# Autodesk Inventor assembly: ABD_MX_64_Roll_Fixation_Set
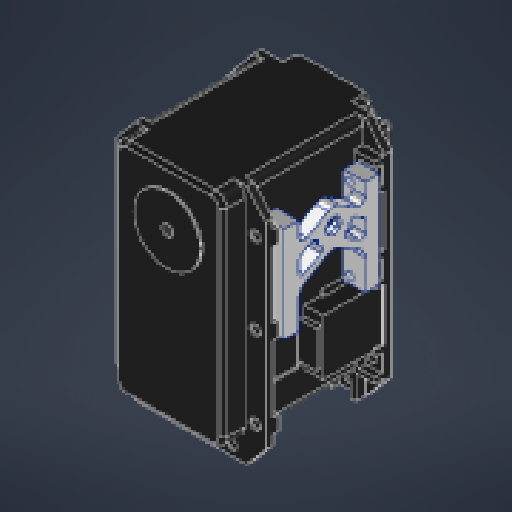
[picture p0: Inventor's stored thumbnail of the model, 512x512]
Saved by Autodesk Inventor 2024.3 (Build 283343000, 343)
## iProperties
Created: 2024-02-15
Part Number: ABD_MX_64_Roll_Fixation_Set
Document SubType Name: Assembly
Designer: ASUS
Author: ASUS
## Documents named in this file (4)
- C:\Users\ASUS\Desktop\Anti_Backlash_Structure_OP\v4_Frame\ABD_MX_64_Roll_Fixation_Set.iam
- C:\Users\ASUS\Desktop\Anti_Backlash_Structure_OP\v4_Frame\Roll_Fixation_L.ipt
- C:\Users\ASUS\Desktop\Anti_Backlash_Structure_OP\v4_Frame\Roll_Fixation_R.ipt
- C:\Users\ASUS\Desktop\Anti_Backlash_Structure_OP\ROBOTIS(Inventor 2024 ver.)\DXL\MX-106T.ipt
## Components (3 placed, 3 different names)
1. Roll_Fixation_R:1 — 플러쉬:1, 메이트:11, 메이트:19
2. Roll_Fixation_L:1 — 플러쉬:1, 메이트:12, 메이트:13, 메이트:14
3. MX-106T:1 — 메이트:11, 메이트:12, 메이트:13, 메이트:14, 메이트:19
## Relationships (6: Mate 5, Flush 1)
- 플러쉬:1 [Flush]: Roll_Fixation_R:1 ↔ Roll_Fixation_L:1
- 메이트:11 [Mate] (0.05 mm): Roll_Fixation_R:1 ↔ MX-106T:1
- 메이트:12 [Mate] (0.05 mm): Roll_Fixation_L:1 ↔ MX-106T:1
- 메이트:13 [Mate]: Roll_Fixation_L:1 ↔ MX-106T:1
- 메이트:14 [Mate]: Roll_Fixation_L:1 ↔ MX-106T:1
- 메이트:19 [Mate]: Roll_Fixation_R:1 ↔ MX-106T:1
